# Autodesk Inventor assembly: CCU_Assembly
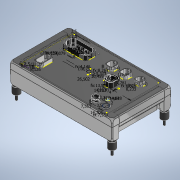
[picture p0: Inventor's stored thumbnail of the model, 180x180]
Saved by Autodesk Inventor 2021 (Build 250183000, 183)
## iProperties
Created: 2020-02-23
Part Number: CCU_Assembly
Document SubType Name: Assembly
Designer: lgnds
Author: lgnds
## Documents named in this file (25)
- C:\Users\Viktor\Documents\GitHub\WaveRunner-CCU\CCU-Assembly\hw\CAD\CCU_Assembly.iam
- C:\Users\Viktor\Documents\GitHub\WaveRunner-CCU\CCU-Assembly\hw\CAD\Box\00126334_BA-281709-F-7024.iam
- C:\Users\Viktor\Documents\GitHub\WaveRunner-CCU\CCU-Assembly\hw\CAD\Box\BA 2817 OT-F.ipt
- C:\Users\Viktor\Documents\GitHub\WaveRunner-CCU\CCU-Assembly\hw\CAD\Connector\c-drc22-50p01-b-3d.ipt
- C:\Users\Viktor\Documents\GitHub\WaveRunner-CCU\CCU-Assembly\hw\CAD\Connector\c-dt15-4p-99-3d.ipt
- C:\Users\Viktor\Documents\GitHub\WaveRunner-CCU\CCU-Assembly\hw\CAD\Connector\c-dt15-6p-99-3d.ipt
- C:\Users\Viktor\Documents\GitHub\WaveRunner-CCU\CCU-Assembly\hw\CAD\Connector\c-dt15-12pa-e-3d.ipt
- C:\Users\Viktor\Documents\GitHub\WaveRunner-CCU\CCU-Assembly\hw\CAD\Connector\c-dtp15-4p-99-3d.ipt
- C:\Users\Viktor\Documents\GitHub\WaveRunner-CCU\CCU-Assembly\hw\CAD\Connector\px0443.iam
- C:\Users\Viktor\Documents\GitHub\WaveRunner-CCU\CCU-Assembly\hw\CAD\Other\82-5151.2123-EAOCorporation--02-23-2020.ipt
- C:\Users\Viktor\Documents\GitHub\WaveRunner-CCU\CCU-Assembly\hw\CAD\Other\LCS_052_XXX_Series.iam
- C:\Users\Viktor\Documents\GitHub\WaveRunner-CCU\CCU-Assembly\hw\CAD\TMCM-1260_PCB.ipt
- C:\Users\Viktor\Documents\GitHub\WaveRunner-CCU\CCU-Assembly\hw\CAD\PlattaAssembly.iam
- C:\Users\Viktor\Documents\GitHub\WaveRunner-CCU\CCU-Assembly\hw\CAD\PCB\TCU_UCU_PCB.ipt
- C:\Users\Viktor\Documents\GitHub\WaveRunner-CCU\CCU-Assembly\hw\CAD\PCB\NCU_PCB.ipt
- C:\Users\Viktor\Documents\GitHub\WaveRunner-CCU\CCU-Assembly\hw\CAD\PCB\ICU_PDU_PCB.ipt
- C:\Users\Viktor\Documents\GitHub\WaveRunner-CCU\CCU-Assembly\hw\CAD\PCB\USB_PROG_PCB.ipt
- C:\Users\Viktor\Documents\GitHub\WaveRunner-CCU\CCU-Assembly\hw\CAD\PCB\LED_PCB.ipt
- C:\Users\Viktor\Documents\GitHub\WaveRunner-CCU\CCU-Assembly\hw\CAD\Other\m300-mv31045m1_asm\m300-mv31045m1_asm.iam
- C:\Users\Viktor\Documents\GitHub\WaveRunner-CCU\CCU-Assembly\hw\CAD\DB2_Bridge_Assembly.iam
- C:\Users\Viktor\Documents\GitHub\WaveRunner-CCU\CCU-Assembly\hw\CAD\Other\MiddleStandOff.ipt
- C:\Users\Viktor\Documents\GitHub\WaveRunner-CCU\CCU-Assembly\hw\CAD\Other\s8131-46r.ipt
- C:\Users\Viktor\Documents\GitHub\WaveRunner-CCU\CCU-Assembly\hw\CAD\Other\Spacer5mm_m3_970050351.ipt
- C:\Users\Viktor\Documents\GitHub\WaveRunner-CCU\CCU-Assembly\hw\CAD\Box\00126324_BA-281706-F-7024.iam
- C:\Users\Viktor\Documents\GitHub\WaveRunner-CCU\CCU-Assembly\hw\CAD\Other\Wiberger-gn451-20-20-m6-es-55.ipt
## Components (40 placed, 24 different names)
1. 00126334_BA-281709-F-7024:1 [sub-assembly] — Flush:1, Flush:2, Mate:1
2. 00126324_BA-281706-F-7024:1 [sub-assembly] — Rotational:3, Rigid:38, Rigid:39, Rigid:40, Rigid:41
3. BA 2817 OT-F:1 — Flush:1, Flush:2, Mate:1, Mate:2, Mate:5, Mate:6, Mate:8, Mate:9, Tangent:1, Tangent:3, Flush:23, Flush:24, Flush:25, Flush:26, Flush:27, Flush:28, Flush:35, Flush:36, Mate:15, Tangent:6, Tangent:7, Flush:39, Flush:40, Mate:18, Rigid:1, Mate:39, Rotational:3
4. c-drc22-50p01-b-3d:1 — Mate:2, Flush:7, Tangent:1, Tangent:3, Flush:23, Flush:24
5. c-dt15-4p-99-3d:1 — Mate:5, Flush:3, Flush:5, Flush:7, Flush:25, Flush:26, Mate:20
6. c-dt15-6p-99-3d:1 — Mate:6, Flush:3, Flush:5, Flush:27, Flush:28, Flush:45, Flush:47
7. c-dt15-12pa-e-3d:1 — Mate:15, Tangent:6, Tangent:7, Flush:39, Flush:40
8. px0443:1 [sub-assembly] — Mate:8, Mate:21, Mate:22
9. LCS_052_XXX_Series:1 [sub-assembly] — Flush:43, Flush:44
10. 82-5151.2123-EAOCorporation--02-23-2020:1 — Mate:9, Flush:35, Flush:36, Mate:23, Mate:24
11. c-dtp15-4p-99-3d:1 — Mate:18, Mate:20, Flush:45, Flush:46
12. PlattaAssembly:1 [sub-assembly] — Rigid:1, Rigid:13, Rigid:14, Rigid:17, Angle:1, Rigid:35, Rigid:36
13. TCU_UCU_PCB:1 — Mate:26, Mate:35, Mate:36, Rigid:23, Rigid:36
14. NCU_PCB:1 — Mate:25, Mate:33, Mate:34, Rigid:14, Rigid:18, Rigid:19, Rigid:20, Rigid:21, Rigid:22, Rigid:30, Rigid:31, Rigid:32, Rigid:33, Angle:1
15. ICU_PDU_PCB:1 — Mate:27, Mate:30, Mate:31, Mate:32, Mate:37, Mate:38
16. USB_PROG_PCB:1 — Rigid:35
17. Spacer5mm_m3_970050351:1 — Rigid:31
18. Spacer5mm_m3_970050351:2 — Rigid:33
19. Spacer5mm_m3_970050351:3 — Rigid:32, Rigid:34
20. Spacer5mm_m3_970050351:4 — Rigid:30
21. LED_PCB:1 — Rigid:13
22. m300-mv31045m1_asm:2 [sub-assembly] — Mate:30, Mate:31, Mate:32, Rotational:2
23. m300-mv31045m1_asm:3 [sub-assembly] — Mate:27, Mate:37, Mate:38, Rigid:11
24. m300-mv31045m1_asm:4 [sub-assembly] — Mate:25, Mate:33, Mate:34
25. m300-mv31045m1_asm:5 [sub-assembly] — Mate:26, Mate:35, Mate:36
26. DB2_Bridge_Assembly:1 [sub-assembly] — Rigid:11
27. DB2_Bridge_Assembly:2 [sub-assembly] — Rotational:2
28. MiddleStandOff:1 — Rigid:17
29. s8131-46r:1 — Rigid:18
30. s8131-46r:2 — Rigid:19
31. s8131-46r:3 — Rigid:21
32. s8131-46r:4 — Rigid:20
33. s8131-46r:5 — Rigid:22
34. s8131-46r:6 — Rigid:23
35. c-dt15-6p-99-3d:2 — Mate:39, Flush:46, Flush:47
36. TMCM-1260_PCB:3 — Rigid:34
37. Wiberger-gn451-20-20-m6-es-55:1 — Rigid:40
38. Wiberger-gn451-20-20-m6-es-55:2 — Rigid:41
39. Wiberger-gn451-20-20-m6-es-55:3 — Rigid:38
40. Wiberger-gn451-20-20-m6-es-55:4 — Rigid:39
## Relationships (76: Mate 27, WeldJoint 22, Flush 20, Tangent 4, RevoluteJoint 2, Angle 1)
- Flush:1: 00126334_BA-281709-F-7024:1 ↔ BA 2817 OT-F:1
- Flush:2: 00126334_BA-281709-F-7024:1 ↔ BA 2817 OT-F:1
- Mate:1: 00126334_BA-281709-F-7024:1 ↔ BA 2817 OT-F:1
- Mate:2: BA 2817 OT-F:1 ↔ c-drc22-50p01-b-3d:1
- Mate:5: BA 2817 OT-F:1 ↔ c-dt15-4p-99-3d:1
- Mate:6: BA 2817 OT-F:1 ↔ c-dt15-6p-99-3d:1
- Mate:8: BA 2817 OT-F:1 ↔ px0443:1
- Mate:9: BA 2817 OT-F:1 ↔ 82-5151.2123-EAOCorporation--02-23-2020:1
- [Mate]: BA 2817 OT-F:1 ↔ LCS_052_XXX_Series:1
- Flush:3 (-80 mm): c-dt15-4p-99-3d:1 ↔ c-dt15-6p-99-3d:1
- Flush:5: c-dt15-4p-99-3d:1 ↔ c-dt15-6p-99-3d:1
- Flush:7: c-drc22-50p01-b-3d:1 ↔ c-dt15-4p-99-3d:1
- Tangent:1 (12.5 mm): BA 2817 OT-F:1 ↔ c-drc22-50p01-b-3d:1
- Tangent:3 (12.5 mm): BA 2817 OT-F:1 ↔ c-drc22-50p01-b-3d:1
- Flush:23: BA 2817 OT-F:1 ↔ c-drc22-50p01-b-3d:1
- Flush:24: BA 2817 OT-F:1 ↔ c-drc22-50p01-b-3d:1
- Flush:25: BA 2817 OT-F:1 ↔ c-dt15-4p-99-3d:1
- Flush:26: BA 2817 OT-F:1 ↔ c-dt15-4p-99-3d:1
- Flush:27: BA 2817 OT-F:1 ↔ c-dt15-6p-99-3d:1
- Flush:28: BA 2817 OT-F:1 ↔ c-dt15-6p-99-3d:1
- Flush:35: BA 2817 OT-F:1 ↔ 82-5151.2123-EAOCorporation--02-23-2020:1
- Flush:36: BA 2817 OT-F:1 ↔ 82-5151.2123-EAOCorporation--02-23-2020:1
- Mate:15: BA 2817 OT-F:1 ↔ c-dt15-12pa-e-3d:1
- Tangent:6 (12.5 mm): BA 2817 OT-F:1 ↔ c-dt15-12pa-e-3d:1
- Tangent:7 (12.5 mm): BA 2817 OT-F:1 ↔ c-dt15-12pa-e-3d:1
- Flush:39: BA 2817 OT-F:1 ↔ c-dt15-12pa-e-3d:1
- Flush:40: BA 2817 OT-F:1 ↔ c-dt15-12pa-e-3d:1
- Mate:18: BA 2817 OT-F:1 ↔ c-dtp15-4p-99-3d:1
- Mate:20 (7 mm): c-dt15-4p-99-3d:1 ↔ c-dtp15-4p-99-3d:1
- Flush:43 (-90 mm): LCS_052_XXX_Series:1
- Flush:44 (40.5 mm): LCS_052_XXX_Series:1
- Mate:21 (75 mm): px0443:1
- Mate:22 (-60 mm): px0443:1
- Mate:23 (-60 mm): 82-5151.2123-EAOCorporation--02-23-2020:1
- Mate:24 (105 mm): 82-5151.2123-EAOCorporation--02-23-2020:1
- Rigid:1 [WeldJoint]: BA 2817 OT-F:1 ↔ PlattaAssembly:1
- Mate:25: NCU_PCB:1 ↔ m300-mv31045m1_asm:4
- Mate:26: TCU_UCU_PCB:1 ↔ m300-mv31045m1_asm:5
- Mate:27: ICU_PDU_PCB:1 ↔ m300-mv31045m1_asm:3
- Mate:30: ICU_PDU_PCB:1 ↔ m300-mv31045m1_asm:2
- Mate:31: ICU_PDU_PCB:1 ↔ m300-mv31045m1_asm:2
- Mate:32: ICU_PDU_PCB:1 ↔ m300-mv31045m1_asm:2
- Mate:33: NCU_PCB:1 ↔ m300-mv31045m1_asm:4
- Mate:34: NCU_PCB:1 ↔ m300-mv31045m1_asm:4
- Mate:35: TCU_UCU_PCB:1 ↔ m300-mv31045m1_asm:5
- Mate:36: TCU_UCU_PCB:1 ↔ m300-mv31045m1_asm:5
- Mate:37: ICU_PDU_PCB:1 ↔ m300-mv31045m1_asm:3
- Mate:38: ICU_PDU_PCB:1 ↔ m300-mv31045m1_asm:3
- Rotational:2 [RevoluteJoint]: m300-mv31045m1_asm:2 ↔ DB2_Bridge_Assembly:2
- Rigid:11 [WeldJoint]: m300-mv31045m1_asm:3 ↔ DB2_Bridge_Assembly:1
- Rigid:13 [WeldJoint]: PlattaAssembly:1 ↔ LED_PCB:1
- Rigid:14 [WeldJoint]: PlattaAssembly:1 ↔ NCU_PCB:1
- Rigid:17 [WeldJoint]: PlattaAssembly:1 ↔ MiddleStandOff:1
- Rigid:18 [WeldJoint]: NCU_PCB:1 ↔ s8131-46r:1
- Rigid:19 [WeldJoint]: NCU_PCB:1 ↔ s8131-46r:2
- Rigid:20 [WeldJoint]: NCU_PCB:1 ↔ s8131-46r:4
- Rigid:21 [WeldJoint]: NCU_PCB:1 ↔ s8131-46r:3
- Rigid:22 [WeldJoint]: NCU_PCB:1 ↔ s8131-46r:5
- Rigid:23 [WeldJoint]: TCU_UCU_PCB:1 ↔ s8131-46r:6
- Flush:45 (-40 mm): c-dt15-6p-99-3d:1 ↔ c-dtp15-4p-99-3d:1
- Mate:39: BA 2817 OT-F:1 ↔ c-dt15-6p-99-3d:2
- Flush:46: c-dtp15-4p-99-3d:1 ↔ c-dt15-6p-99-3d:2
- Flush:47: c-dt15-6p-99-3d:1 ↔ c-dt15-6p-99-3d:2
- Rigid:30 [WeldJoint]: NCU_PCB:1 ↔ Spacer5mm_m3_970050351:4
- Rigid:31 [WeldJoint]: NCU_PCB:1 ↔ Spacer5mm_m3_970050351:1
- Rigid:32 [WeldJoint]: NCU_PCB:1 ↔ Spacer5mm_m3_970050351:3
- Rigid:33 [WeldJoint]: NCU_PCB:1 ↔ Spacer5mm_m3_970050351:2
- Rigid:34 [WeldJoint]: Spacer5mm_m3_970050351:3 ↔ TMCM-1260_PCB:3
- Angle:1 (0 deg): PlattaAssembly:1 ↔ NCU_PCB:1
- Rigid:35 [WeldJoint]: PlattaAssembly:1 ↔ USB_PROG_PCB:1
- Rigid:36 [WeldJoint]: PlattaAssembly:1 ↔ TCU_UCU_PCB:1
- Rotational:3 [RevoluteJoint]: 00126324_BA-281706-F-7024:1 ↔ BA 2817 OT-F:1
- Rigid:38 [WeldJoint]: 00126324_BA-281706-F-7024:1 ↔ Wiberger-gn451-20-20-m6-es-55:3
- Rigid:39 [WeldJoint]: 00126324_BA-281706-F-7024:1 ↔ Wiberger-gn451-20-20-m6-es-55:4
- Rigid:40 [WeldJoint]: 00126324_BA-281706-F-7024:1 ↔ Wiberger-gn451-20-20-m6-es-55:1
- Rigid:41 [WeldJoint]: 00126324_BA-281706-F-7024:1 ↔ Wiberger-gn451-20-20-m6-es-55:2
